# Autodesk Inventor assembly: Tarraxa
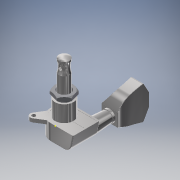
[picture p0: Inventor's stored thumbnail of the model, 180x180]
Saved by Autodesk Inventor 2016 (Build 200138000, 138)
## iProperties
Created: 2018-12-06
Part Number: Tarraxa
Document SubType Name: Assembly
Designer: dqm_r
Author: dqm_r
## Documents named in this file (5)
- C:\Users\dqm_r\OneDrive\Documentos\Inventor\Guitarra\Tarraxa.iam
- C:\Users\dqm_r\OneDrive\Documentos\Inventor\Guitarra\Peça 7.ipt
- C:\Users\dqm_r\OneDrive\Documentos\Inventor\Guitarra\Cabeça da tarraxa.ipt
- C:\Users\dqm_r\OneDrive\Documentos\Inventor\Guitarra\Parafuso menor Tarraxa.ipt
- C:\Users\dqm_r\OneDrive\Documentos\Inventor\Guitarra\Parafuso Tarraxa.ipt
## Components (4 placed, 4 different names)
1. Peça 7:1 — Mate:1, Rotational:1, Cylindrical:1
2. Cabeça da tarraxa:1 — Mate:1, Rotational:1, Insert:1
3. Parafuso menor Tarraxa:1 — Insert:1
4. Parafuso Tarraxa:1 — Cylindrical:1
## Relationships (4: Mate 1, RevoluteJoint 1, Insert 1, CylindricalJoint 1)
- Mate:1: Peça 7:1 ↔ Cabeça da tarraxa:1
- Rotational:1 [RevoluteJoint]: Peça 7:1 ↔ Cabeça da tarraxa:1
- Insert:1: Cabeça da tarraxa:1 ↔ Parafuso menor Tarraxa:1
- Cylindrical:1: Peça 7:1 ↔ Parafuso Tarraxa:1
